# Autodesk Inventor assembly: walls
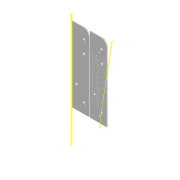
[picture p0: Inventor's stored thumbnail of the model, 180x180]
Saved by Autodesk Inventor 2020 (Build 240168000, 168)
## iProperties
Created: 2019-11-20
Part Number: walls
Document SubType Name: Assembly
Designer: ball
Author: ball
## Documents named in this file (3)
- C:\FTC\FTC8863CAD\2019 Robot\Mecanum Drive Train\walls.iam
- C:\FTC\FTC8863CAD\2019 Robot\Mecanum Drive Train\inside wall.ipt
- C:\FTC\FTC8863CAD\2019 Robot\Mecanum Drive Train\outside wall.ipt
## Components (2 placed, 2 different names)
1. inside wall:1 — Mate:1, Flush:1, Flush:2
2. outside wall:1 — Mate:1, Flush:1, Flush:2
## Relationships (3: Flush 2, Mate 1)
- Mate:1 (6.35 mm): inside wall:1 ↔ outside wall:1
- Flush:1: inside wall:1 ↔ outside wall:1
- Flush:2: inside wall:1 ↔ outside wall:1
